# Autodesk Inventor assembly: innerhub_assembly
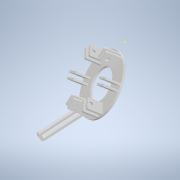
[picture p0: Inventor's stored thumbnail of the model, 180x180]
Saved by Autodesk Inventor 2020 (Build 240168000, 168)
## iProperties
Created: 2019-09-23
Part Number: innerhub_assembly
Document SubType Name: Assembly
Designer: dlr6513
Author: dlr6513
## Documents named in this file (4)
- C:\Users\dlr6513\Documents\eli_inventor_practice\innerhub_assembly.iam
- C:\Users\dlr6513\Documents\eli_inventor_practice\inner_hub.ipt
- C:\Users\dlr6513\Documents\eli_inventor_practice\extention_plate.ipt
- C:\Users\dlr6513\Documents\eli_inventor_practice\extention_rod.ipt
## Components (3 placed, 3 different names)
1. inner_hub:1 — Flush:1, Flush:2, Flush:3, Tangent:1, Mate:1
2. extention_plate:1 — Mate:1
3. extention_rod:1 — Flush:1, Flush:2, Flush:3, Tangent:1
## Relationships (5: Flush 3, Tangent 1, Mate 1)
- Flush:1: inner_hub:1 ↔ extention_rod:1
- Flush:2: inner_hub:1 ↔ extention_rod:1
- Flush:3: inner_hub:1 ↔ extention_rod:1
- Tangent:1: inner_hub:1 ↔ extention_rod:1
- Mate:1: inner_hub:1 ↔ extention_plate:1
